# Autodesk Inventor assembly: FULL FINGE6
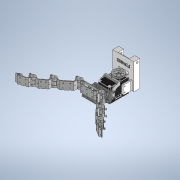
[picture p0: Inventor's stored thumbnail of the model, 180x180]
Saved by Autodesk Inventor 2021 (Build 250183000, 183)
## iProperties
Created: 2022-10-03
Part Number: FULL FINGE6
Document SubType Name: Assembly
Designer: ereg140
Author: ereg140
## Documents named in this file (10)
- \\files.auckland.ac.nz\myhome\Documents\GitHub\hand\FULL FINGE6.iam
- \\files.auckland.ac.nz\myhome\Documents\GitHub\hand\XM430 Motor\XM430-Working-Shaft.iam
- \\files.auckland.ac.nz\myhome\Documents\GitHub\hand\Pully_smlaller.ipt
- \\files.auckland.ac.nz\myhome\Documents\GitHub\hand\Dovetail\dovetail_female_Dyna_Mount.ipt
- \\files.auckland.ac.nz\myhome\Documents\GitHub\hand\Dynamixel_Palm_Bracket_2.ipt
- \\files.auckland.ac.nz\myhome\Documents\GitHub\hand\Tendon_Center.ipt
- \\files.auckland.ac.nz\myhome\Documents\GitHub\hand\FINGIE_6_palm_50mm.ipt
- \\files.auckland.ac.nz\myhome\Documents\GitHub\hand\Phalalnge6_35mm_TIP_hdm.ipt
- \\files.auckland.ac.nz\myhome\Documents\GitHub\hand\Phalalnge6_HDM_35mm.ipt
- \\files.auckland.ac.nz\myhome\Documents\GitHub\hand\Phalalnge6_HDM_42mm.ipt
## Components (12 placed, 9 different names)
1. XM430-Working-Shaft:1 [sub-assembly] — Angle:1, Rigid:4, Mate:1, Mate:2, Slider:1, Rigid:7, Rigid:8
2. Pully_smlaller:1 — Rigid:4
3. dovetail_female_Dyna_Mount:1 — Mate:1, Mate:2, Slider:1
4. Dynamixel_Palm_Bracket_2:1 — Rigid:7, Rigid:9
5. Tendon_Center:1 — Rigid:8
6. FINGIE_6_palm_50mm:1 — Rigid:9, Planar:1, Planar:2, Planar:3, Cylindrical:1, Planar:4, Cylindrical:4
7. Phalalnge6_35mm_TIP_hdm:1 — Planar:3, Cylindrical:6
8. Phalalnge6_HDM_35mm:1 — Planar:2, Cylindrical:5, Cylindrical:6
9. Phalalnge6_HDM_42mm:1 — Planar:1, Cylindrical:4, Cylindrical:5
10. Phalalnge6_35mm_TIP_hdm:2 — Cylindrical:3, Planar:6
11. Phalalnge6_HDM_35mm:2 — Cylindrical:2, Cylindrical:3, Planar:5, Planar:6
12. Phalalnge6_HDM_42mm:2 — Cylindrical:1, Cylindrical:2, Planar:4, Planar:5
## Relationships (20: PlanarJoint 6, CylindricalJoint 6, WeldJoint 4, Mate 2, Angle 1, TranslationJoint 1)
- Angle:1 (0 deg): XM430-Working-Shaft:1
- Rigid:4 [WeldJoint]: XM430-Working-Shaft:1 ↔ Pully_smlaller:1
- Mate:1: XM430-Working-Shaft:1 ↔ dovetail_female_Dyna_Mount:1
- Mate:2: XM430-Working-Shaft:1 ↔ dovetail_female_Dyna_Mount:1
- Slider:1 [TranslationJoint]: XM430-Working-Shaft:1 ↔ dovetail_female_Dyna_Mount:1
- Rigid:7 [WeldJoint]: XM430-Working-Shaft:1 ↔ Dynamixel_Palm_Bracket_2:1
- Rigid:8 [WeldJoint]: XM430-Working-Shaft:1 ↔ Tendon_Center:1
- Rigid:9 [WeldJoint]: Dynamixel_Palm_Bracket_2:1 ↔ FINGIE_6_palm_50mm:1
- Planar:1: FINGIE_6_palm_50mm:1 ↔ Phalalnge6_HDM_42mm:1
- Planar:2: FINGIE_6_palm_50mm:1 ↔ Phalalnge6_HDM_35mm:1
- Planar:3: FINGIE_6_palm_50mm:1 ↔ Phalalnge6_35mm_TIP_hdm:1
- Cylindrical:1: FINGIE_6_palm_50mm:1 ↔ Phalalnge6_HDM_42mm:2
- Cylindrical:2: Phalalnge6_HDM_35mm:2 ↔ Phalalnge6_HDM_42mm:2
- Cylindrical:3: Phalalnge6_35mm_TIP_hdm:2 ↔ Phalalnge6_HDM_35mm:2
- Planar:4: FINGIE_6_palm_50mm:1 ↔ Phalalnge6_HDM_42mm:2
- Planar:5: Phalalnge6_HDM_35mm:2 ↔ Phalalnge6_HDM_42mm:2
- Planar:6: Phalalnge6_35mm_TIP_hdm:2 ↔ Phalalnge6_HDM_35mm:2
- Cylindrical:4: FINGIE_6_palm_50mm:1 ↔ Phalalnge6_HDM_42mm:1
- Cylindrical:5: Phalalnge6_HDM_35mm:1 ↔ Phalalnge6_HDM_42mm:1
- Cylindrical:6: Phalalnge6_35mm_TIP_hdm:1 ↔ Phalalnge6_HDM_35mm:1
## Named parameters: sa_0 = 30000
note: some values were not read from the file. Shown as the stored number, unit unknown: "sa_0".
